# Autodesk Inventor assembly: клешня сбора
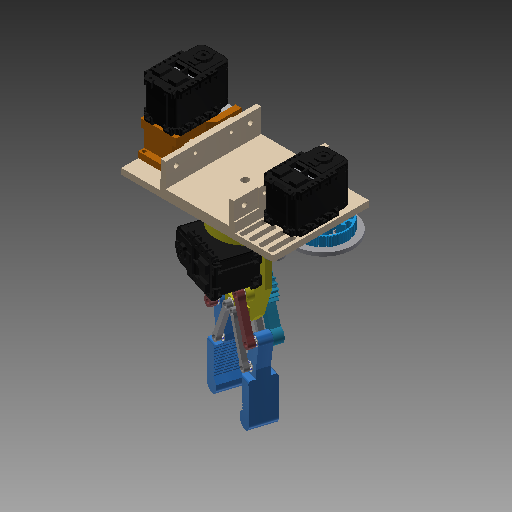
[picture p0: Inventor's stored thumbnail of the model, 512x512]
Saved by Autodesk Inventor 2019 (Build 230136000, 136)
## iProperties
Created: 2019-08-15
Part Number: клешня сбора
Material: Типовые
Document SubType Name: Assembly
Designer: Петров Иван
Mass: 355.856 g
Surface Area: 1411.74 cm^2
Volume: 301.215 cm^3
Density: 1.1814 g/cm^3
Author: Петров Иван
## Documents named in this file (10)
- E:\IVAN\Ivan_desktop\Kvantorium\Projects\optimal_gripper\hardware\КВ33.044.100 - Захват.iam
- E:\IVAN\Ivan_desktop\Kvantorium\Projects\optimal_gripper\hardware\КВ33.044.101 - Опора захвата.ipt
- E:\IVAN\Ivan_desktop\Kvantorium\Projects\optimal_gripper\hardware\Стандартные изделия\Сервомотор Dynamixel AX-12A\AX-12.iam
- E:\IVAN\Ivan_desktop\Kvantorium\Projects\optimal_gripper\hardware\Стандартные изделия\Проставка 4 мм.ipt
- E:\IVAN\Ivan_desktop\Kvantorium\Projects\optimal_gripper\hardware\Стандартные изделия\Шкив большой Makeblock.ipt
- E:\IVAN\Ivan_desktop\Kvantorium\Projects\optimal_gripper\hardware\Стандартные изделия\Боковина шкива уменьшанная.ipt
- E:\IVAN\Ivan_desktop\Kvantorium\Projects\optimal_gripper\hardware\Стандартные изделия\Шкив большой сборка.iam
- E:\IVAN\Ivan_desktop\Kvantorium\Projects\optimal_gripper\hardware\КВ33.044.200 - Сборка зажима.iam
- E:\IVAN\Ivan_desktop\Kvantorium\Projects\optimal_gripper\hardware\Стандартные изделия\Шкив плоский Makeblock сборка.iam
- E:\IVAN\Ivan_desktop\Kvantorium\Projects\optimal_gripper\hardware\КВ33.044.900 - Клапан присоски впускной.iam
## Components (9 placed, 9 different names)
1. КВ33.044.101 - Опора захвата:1 — Совмещение:17, Совмещение:18, Совмещение:25, Касательность:1, Касательность:2, Совмещение:28, Совмещение:29, Совмещение:30, Совмещение:31, Совмещение:32, Совмещение:33
2. AX-12:1 [sub-assembly] — Совмещение:31, Совмещение:32, Совмещение:33, Совмещение:34, Совмещение:35
3. Проставка 4 мм:1 — Совмещение:6, Совмещение:7, Совмещение:8, Совмещение:34
4. Шкив большой Makeblock:1 — Совмещение:6, Совмещение:7, Совмещение:8, Совмещение:14, Совмещение:15, Совмещение:16, Направление навивки:1
5. Боковина шкива уменьшанная:1 — Совмещение:14, Совмещение:15, Совмещение:16, Совмещение:35, Направление навивки:2
6. Шкив большой сборка:1 [sub-assembly] — Совмещение:17, Совмещение:18, Направление навивки:1, Совмещение:36, Совмещение:37, Совмещение:38
7. КВ33.044.200 - Сборка зажима:1 [sub-assembly] — Совмещение:36, Совмещение:37, Совмещение:38
8. Шкив плоский Makeblock сборка:1 [sub-assembly] — Совмещение:25, Касательность:1, Касательность:2, Направление навивки:2
9. КВ33.044.900 - Клапан присоски впускной:1 [sub-assembly] — Совмещение:28, Совмещение:29, Совмещение:30
## Relationships (24: Mate 20, RelateRotation 2, Tangent 2)
- Совмещение:6 [Mate]: Проставка 4 мм:1 ↔ Шкив большой Makeblock:1
- Совмещение:7 [Mate]: Проставка 4 мм:1 ↔ Шкив большой Makeblock:1
- Совмещение:8 [Mate]: Проставка 4 мм:1 ↔ Шкив большой Makeblock:1
- Совмещение:14 [Mate]: Шкив большой Makeblock:1 ↔ Боковина шкива уменьшанная:1
- Совмещение:15 [Mate]: Шкив большой Makeblock:1 ↔ Боковина шкива уменьшанная:1
- Совмещение:16 [Mate]: Шкив большой Makeblock:1 ↔ Боковина шкива уменьшанная:1
- Совмещение:17 [Mate] (4.24 mm): КВ33.044.101 - Опора захвата:1 ↔ Шкив большой сборка:1
- Совмещение:18 [Mate]: КВ33.044.101 - Опора захвата:1 ↔ Шкив большой сборка:1
- Направление навивки:1 [RelateRotation] (1 ul): Шкив большой Makeblock:1 ↔ Шкив большой сборка:1
- Совмещение:25 [Mate]: КВ33.044.101 - Опора захвата:1 ↔ Шкив плоский Makeblock сборка:1
- Касательность:1 [Tangent]: КВ33.044.101 - Опора захвата:1 ↔ Шкив плоский Makeblock сборка:1
- Касательность:2 [Tangent]: КВ33.044.101 - Опора захвата:1 ↔ Шкив плоский Makeblock сборка:1
- Совмещение:28 [Mate]: КВ33.044.101 - Опора захвата:1 ↔ КВ33.044.900 - Клапан присоски впускной:1
- Совмещение:29 [Mate]: КВ33.044.101 - Опора захвата:1 ↔ КВ33.044.900 - Клапан присоски впускной:1
- Совмещение:30 [Mate]: КВ33.044.101 - Опора захвата:1 ↔ КВ33.044.900 - Клапан присоски впускной:1
- Совмещение:31 [Mate]: КВ33.044.101 - Опора захвата:1 ↔ AX-12:1
- Совмещение:32 [Mate]: КВ33.044.101 - Опора захвата:1 ↔ AX-12:1
- Совмещение:33 [Mate]: КВ33.044.101 - Опора захвата:1 ↔ AX-12:1
- Совмещение:34 [Mate]: AX-12:1 ↔ Проставка 4 мм:1
- Совмещение:35 [Mate]: AX-12:1 ↔ Боковина шкива уменьшанная:1
- Направление навивки:2 [RelateRotation] (0.2 ul): Боковина шкива уменьшанная:1 ↔ Шкив плоский Makeblock сборка:1
- Совмещение:36 [Mate]: Шкив большой сборка:1 ↔ КВ33.044.200 - Сборка зажима:1
- Совмещение:37 [Mate]: Шкив большой сборка:1 ↔ КВ33.044.200 - Сборка зажима:1
- Совмещение:38 [Mate]: Шкив большой сборка:1 ↔ КВ33.044.200 - Сборка зажима:1
